# Autodesk Inventor assembly: Motors Full Assembly
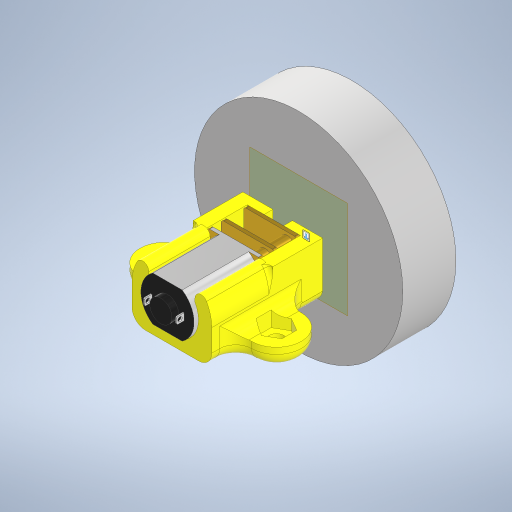
[picture p0: Inventor's stored thumbnail of the model, 512x512]
Saved by Autodesk Inventor 2023 (Build 270158000, 158)
## iProperties
Created: 2023-10-05
Part Number: Motors Full Assembly
Document SubType Name: Assembly
Designer: say514
Author: say514
## Documents named in this file (4)
- H:\Year 3 Tasks\Motors Full Assembly.iam
- H:\Year 3 Tasks\MotorHolder.ipt
- H:\Year 3 Tasks\Pololu_MMG_Motor.ipt
- H:\Year 3 Tasks\Wheel.ipt
## Components (3 placed, 3 different names)
1. MotorHolder:1 — Mate:1, Mate:2, Mate:3
2. Pololu_MMG_Motor:1 — Mate:1, Mate:2, Mate:3, Insert:1
3. Wheel:1 — Insert:1
## Relationships (4: Mate 3, Insert 1)
- Mate:1: MotorHolder:1 ↔ Pololu_MMG_Motor:1
- Mate:2: MotorHolder:1 ↔ Pololu_MMG_Motor:1
- Mate:3: MotorHolder:1 ↔ Pololu_MMG_Motor:1
- Insert:1 (-6 mm): Pololu_MMG_Motor:1 ↔ Wheel:1
